# Autodesk Inventor assembly: Bracing
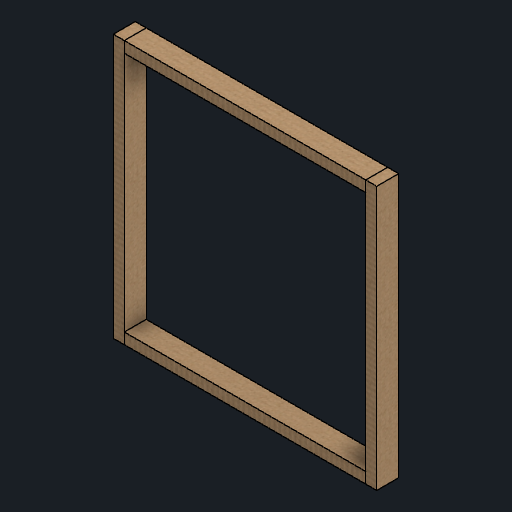
[picture p0: Inventor's stored thumbnail of the model, 512x512]
Saved by Autodesk Inventor 2026.2 (Build 302298000, 298)
## iProperties
Created: 2026-06-19
Part Number: Bracing
Document SubType Name: Assembly
Designer: JoshuaEah
Author: JoshuaEah
## Documents named in this file (3)
- C:\Users\JoshuaEah\Documents\GitHub\Designed-Trinkets\Guitar\110 Guitar Cab\Bracing.iam
- C:\Users\JoshuaEah\Documents\GitHub\Designed-Trinkets\Guitar\110 Guitar Cab\12in Brace.ipt
- C:\Users\JoshuaEah\Documents\GitHub\Designed-Trinkets\Guitar\110 Guitar Cab\11in Brace.ipt
## Components (4 placed, 2 different names)
1. 12in Brace:1
2. 12in Brace:2
3. 11in Brace:1
4. 11in Brace:2
## Relationships (6: Flush 4, Mate 2)
- [Mate]: 12in Brace:1 ↔ 11in Brace:1
- [Flush]: 12in Brace:1 ↔ 11in Brace:1
- [Flush]: 12in Brace:1 ↔ 11in Brace:1
- [Mate]: 12in Brace:1 ↔ 11in Brace:2
- [Flush]: 12in Brace:1 ↔ 11in Brace:2
- [Flush]: 12in Brace:1 ↔ 11in Brace:2
